# Autodesk Inventor assembly: Tapicerka_siedziska
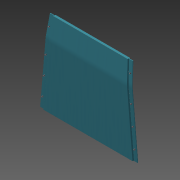
[picture p0: Inventor's stored thumbnail of the model, 180x180]
Saved by Autodesk Inventor 2015 (Build 190159000, 159)
## iProperties
Created: 2015-12-07
Part Number: Tapicerka_siedziska
Document SubType Name: Assembly
Designer: graaapsik
Author: graaapsik
## Documents named in this file (7)
- C:\Users\EriveltonDell\Documents\Centro Universitário da FEI\Wheelchair\CADEIRA DE RODAS - DESENHO\Model\Tapicerka_siedziska.iam
- C:\Users\EriveltonDell\Documents\Centro Universitário da FEI\Wheelchair\CADEIRA DE RODAS - DESENHO\Model\Pianka_siedziska.ipt
- C:\Users\EriveltonDell\Documents\Centro Universitário da FEI\Wheelchair\CADEIRA DE RODAS - DESENHO\Model\Tapicerka_siedziska.ipt
- C:\Users\EriveltonDell\Documents\Centro Universitário da FEI\Wheelchair\CADEIRA DE RODAS - DESENHO\Model\Listwa_siedziska_lewa.ipt
- C:\Users\EriveltonDell\Documents\Centro Universitário da FEI\Wheelchair\CADEIRA DE RODAS - DESENHO\Model\Listwa_siedziska_prawa.ipt
- C:\Users\EriveltonDell\Documents\Centro Universitário da FEI\Wheelchair\CADEIRA DE RODAS - DESENHO\Model\ISO 7092 - ST 6 - 140 HV.ipt
- C:\Users\EriveltonDell\Documents\Centro Universitário da FEI\Wheelchair\CADEIRA DE RODAS - DESENHO\Model\ISO 7380 - M6 x 10.ipt
## Components (20 placed, 6 different names)
1. Tapicerka_siedziska:1 — Zestawiający:1, Zestawiający:2, Równoległy:1, Równoległy:2, Równoległy:3, Równoległy:4, Równoległy:5, Wstaw:1, Wstaw:2, Wstaw:3, Wstaw:4, Wstaw:5, Wstaw:6, Wstaw:7, Wstaw:8, Równoległy:6
2. Pianka_siedziska:1 — Zestawiający:1, Zestawiający:2, Równoległy:1
3. Listwa_siedziska_lewa:1 — Równoległy:3, Równoległy:4, Równoległy:5
4. Listwa_siedziska_prawa:1 — Równoległy:2
5. ISO 7092 ST 6 - 140 HV:1 — Wstaw:1, Wstaw:16
6. ISO 7092 ST 6 - 140 HV:2 — Wstaw:2, Zestawiający:5, Zestawiający:6
7. ISO 7092 ST 6 - 140 HV:3 — Wstaw:3, Wstaw:17
8. ISO 7092 ST 6 - 140 HV:4 — Wstaw:4, Wstaw:21
9. ISO 7092 ST 6 - 140 HV:5 — Wstaw:5, Wstaw:22
10. ISO 7092 ST 6 - 140 HV:6 — Wstaw:6, Wstaw:20
11. ISO 7092 ST 6 - 140 HV:7 — Wstaw:7, Wstaw:18
12. ISO 7092 ST 6 - 140 HV:8 — Wstaw:8, Wstaw:19
13. ISO 7380 M6 x 10:9 — Wstaw:16
14. ISO 7380 M6 x 10:10 — Zestawiający:5, Zestawiający:6
15. ISO 7380 M6 x 10:11 — Wstaw:17
16. ISO 7380 M6 x 10:12 — Wstaw:18
17. ISO 7380 M6 x 10:13 — Wstaw:19
18. ISO 7380 M6 x 10:14 — Wstaw:20
19. ISO 7380 M6 x 10:15 — Wstaw:21
20. ISO 7380 M6 x 10:16 — Wstaw:22
## Relationships (25: Insert 15, Flush 6, Mate 4)
- Zestawiający:1 [Mate] (0.25 mm): Tapicerka_siedziska:1 ↔ Pianka_siedziska:1
- Zestawiający:2 [Mate] (-0.25 mm): Tapicerka_siedziska:1 ↔ Pianka_siedziska:1
- Równoległy:1 [Flush] (-21 mm): Tapicerka_siedziska:1 ↔ Pianka_siedziska:1
- Równoległy:2 [Flush] (-0.55 mm): Tapicerka_siedziska:1 ↔ Listwa_siedziska_prawa:1
- Równoległy:3 [Flush] (0.55 mm): Tapicerka_siedziska:1 ↔ Listwa_siedziska_lewa:1
- Równoległy:4 [Flush] (0.55 mm): Tapicerka_siedziska:1 ↔ Listwa_siedziska_lewa:1
- Równoległy:5 [Flush] (-0.55 mm): Tapicerka_siedziska:1 ↔ Listwa_siedziska_lewa:1
- Wstaw:1 [Insert]: Tapicerka_siedziska:1 ↔ ISO 7092 ST 6 - 140 HV:1
- Wstaw:2 [Insert]: Tapicerka_siedziska:1 ↔ ISO 7092 ST 6 - 140 HV:2
- Wstaw:3 [Insert]: Tapicerka_siedziska:1 ↔ ISO 7092 ST 6 - 140 HV:3
- Wstaw:4 [Insert]: Tapicerka_siedziska:1 ↔ ISO 7092 ST 6 - 140 HV:4
- Wstaw:5 [Insert]: Tapicerka_siedziska:1 ↔ ISO 7092 ST 6 - 140 HV:5
- Wstaw:6 [Insert]: Tapicerka_siedziska:1 ↔ ISO 7092 ST 6 - 140 HV:6
- Wstaw:7 [Insert]: Tapicerka_siedziska:1 ↔ ISO 7092 ST 6 - 140 HV:7
- Wstaw:8 [Insert]: Tapicerka_siedziska:1 ↔ ISO 7092 ST 6 - 140 HV:8
- Równoległy:6 [Flush] (224.25 mm): Tapicerka_siedziska:1
- Wstaw:16 [Insert]: ISO 7092 ST 6 - 140 HV:1 ↔ ISO 7380 M6 x 10:9
- Zestawiający:5 [Mate]: ISO 7092 ST 6 - 140 HV:2 ↔ ISO 7380 M6 x 10:10
- Zestawiający:6 [Mate]: ISO 7092 ST 6 - 140 HV:2 ↔ ISO 7380 M6 x 10:10
- Wstaw:17 [Insert]: ISO 7092 ST 6 - 140 HV:3 ↔ ISO 7380 M6 x 10:11
- Wstaw:18 [Insert]: ISO 7092 ST 6 - 140 HV:7 ↔ ISO 7380 M6 x 10:12
- Wstaw:19 [Insert]: ISO 7092 ST 6 - 140 HV:8 ↔ ISO 7380 M6 x 10:13
- Wstaw:20 [Insert]: ISO 7092 ST 6 - 140 HV:6 ↔ ISO 7380 M6 x 10:14
- Wstaw:21 [Insert]: ISO 7092 ST 6 - 140 HV:4 ↔ ISO 7380 M6 x 10:15
- Wstaw:22 [Insert]: ISO 7092 ST 6 - 140 HV:5 ↔ ISO 7380 M6 x 10:16
